# Autodesk Inventor assembly: ASY GBK 2130 short wall shield 3
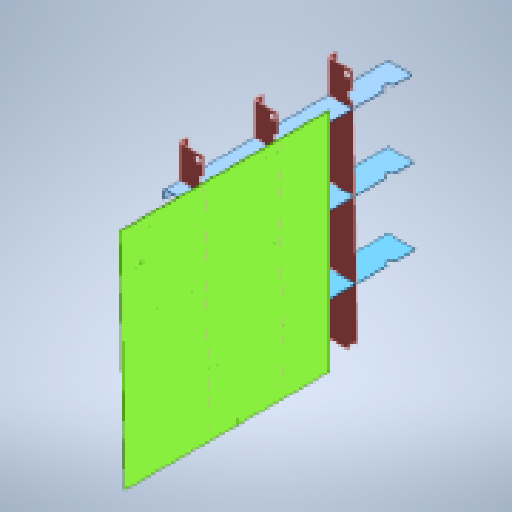
[picture p0: Inventor's stored thumbnail of the model, 512x512]
Saved by Autodesk Inventor 2026 (Build 300175000, 175)
## iProperties
Created: 2026-05-07
Part Number: ASY GBK 2130 short wall shield 3
Document SubType Name: Assembly
Designer: pokla
Stock Number: 1111
Mass: 136093 g
Surface Area: 87957.2 cm^2
Volume: 17336.7 cm^3
Density: 7.85 g/cm^3
Author: admin
## Documents named in this file (6)
- C:\Users\pokla\Documents\Inventor\GBK-Gubkinskiy\ASY GBK 2130 short wall shield 3.iam
- C:\Users\pokla\Documents\Inventor\GBK-Gubkinskiy\GBK 0101 main rib.ipt
- C:\Users\pokla\Documents\Inventor\GBK-Gubkinskiy\GBK 0102 stringer 1.ipt
- C:\Users\pokla\Documents\Inventor\GBK-Gubkinskiy\GBK 0103 stringer 2.ipt
- C:\Users\pokla\Documents\Inventor\GBK-Gubkinskiy\GBK 0104 stringer 3.ipt
- C:\Users\pokla\Documents\Inventor\GBK-Gubkinskiy\GBK 2133 shield 3.ipt
## Components (7 placed, 5 different names)
1. GBK 0101 main rib.ipt:1 — Совмещение:3, Совмещение:5, Жесткий:1, Жесткий:2, Жесткий:3, Совмещение:5
2. GBK 0102 stringer 1.ipt:1 — Жесткий:1, Жесткий:4, Жесткий:5
3. GBK 0103 stringer 2.ipt:1 — Жесткий:2, Заподлицо:2
4. GBK 0104 stringer 3.ipt:1 — Жесткий:3
5. GBK 0101 main rib.ipt:2 — Жесткий:4
6. GBK 0101 main rib.ipt:3 — Жесткий:5
7. GBK 2133 shield 3.ipt:1 — Заподлицо:1, Совмещение:5, Совмещение:6, Заподлицо:2
## Relationships (11: WeldJoint 5, Mate 4, Flush 2)
- Совмещение:3 [Mate]: GBK 0101 main rib.ipt:1
- Совмещение:5 [Mate]: GBK 0101 main rib.ipt:1
- Жесткий:1 [WeldJoint] (4 mm): GBK 0101 main rib.ipt:1 ↔ GBK 0102 stringer 1.ipt:1
- Жесткий:2 [WeldJoint] (4 mm): GBK 0101 main rib.ipt:1 ↔ GBK 0103 stringer 2.ipt:1
- Жесткий:3 [WeldJoint] (4 mm): GBK 0101 main rib.ipt:1 ↔ GBK 0104 stringer 3.ipt:1
- Жесткий:4 [WeldJoint] (4 mm): GBK 0102 stringer 1.ipt:1 ↔ GBK 0101 main rib.ipt:2
- Жесткий:5 [WeldJoint] (4 mm): GBK 0102 stringer 1.ipt:1 ↔ GBK 0101 main rib.ipt:3
- Заподлицо:1 [Flush]: GBK 2133 shield 3.ipt:1
- Совмещение:5 [Mate]: GBK 0101 main rib.ipt:1 ↔ GBK 2133 shield 3.ipt:1
- Совмещение:6 [Mate]: GBK 2133 shield 3.ipt:1
- Заподлицо:2 [Flush] (155 mm): GBK 0103 stringer 2.ipt:1 ↔ GBK 2133 shield 3.ipt:1
